# Autodesk Inventor assembly: P1704_E001
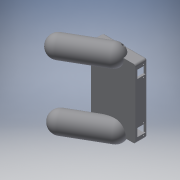
[picture p0: Inventor's stored thumbnail of the model, 180x180]
Saved by Autodesk Inventor 2019 (Build 230136000, 136)
## iProperties
Created: 2019-04-29
Part Number: P1704_E001
Material: Générique
Document SubType Name: Assembly
Designer: Joan.MAILLARD
Author: Joan.MAILLARD
## Documents named in this file (4)
- P:\projet_manette\manette\06_Dessins\P1704_E001.iam
- P:\projet_manette\manette\06_Dessins\P1704_002_mainDroite.ipt
- P:\projet_manette\manette\06_Dessins\P1704_003_mainGauche.ipt
- P:\projet_manette\manette\06_Dessins\P1794_001_basManette.ipt
## Components (3 placed, 3 different names)
1. P1704_002_mainDroite:1 — Rotation:1
2. P1704_003_mainGauche:1 — Rotation:2
3. P1794_001_basManette:1 — Rotation:1, Rotation:2
## Relationships (2: RevoluteJoint 2)
- Rotation:1 [RevoluteJoint]: P1704_002_mainDroite:1 ↔ P1794_001_basManette:1
- Rotation:2 [RevoluteJoint]: P1704_003_mainGauche:1 ↔ P1794_001_basManette:1
